# Autodesk Inventor assembly: New_Case
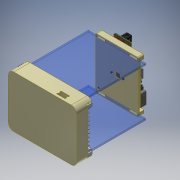
[picture p0: Inventor's stored thumbnail of the model, 180x180]
Saved by Autodesk Inventor 2017 (Build 210142000, 142)
## iProperties
Created: 2017-11-02
Part Number: New_Case
Document SubType Name: Assembly
Designer: P. Baesso
Author: P. Baesso
## Documents named in this file (16)
- E:\Rymapt_projects\Ethoscope\ethoscope_hardware\Assembled\New_Case.iam
- E:\Rymapt_projects\Ethoscope\ethoscope_hardware\core\RPi3\RPi3_ModelB.ipt
- E:\Rymapt_projects\Ethoscope\ethoscope_hardware\core_Rymapt\PiCase\lowerPiCase_small.ipt
- E:\Rymapt_projects\Ethoscope\ethoscope_hardware\core\RPi3\RasPi_Camera.ipt
- E:\Rymapt_projects\Ethoscope\ethoscope_hardware\Shield\Files\PCB_R2D2.iam
- E:\Rymapt_projects\Ethoscope\ethoscope_hardware\core_Rymapt\PiCase\upperPiCase_small.ipt
- E:\Rymapt_projects\Ethoscope\ethoscope_hardware\core_Rymapt\LightBox\sideWall_R3.ipt
- E:\Rymapt_projects\Ethoscope\ethoscope_hardware\extra\IRFilter\FB700-10-Step.ipt
- E:\Rymapt_projects\Ethoscope\ethoscope_hardware\extra\IRFilter\FilterHolder.ipt
- E:\Rymapt_projects\Ethoscope\ethoscope_hardware\core_Rymapt\LightBox\core_lightBox_R2.ipt
- E:\Rymapt_projects\Ethoscope\ethoscope_hardware\core_Rymapt\LightBox\core_lightStrip_R.ipt
- E:\Rymapt_projects\Ethoscope\ethoscope_hardware\arenas\arena_10x1_longTubes\arena_10x1_longTubes.ipt
- E:\Rymapt_projects\Ethoscope\ethoscope_hardware\extra\Screws\SpacerShiel.ipt
- E:\Rymapt_projects\Ethoscope\ethoscope_hardware\extra\Screws\M2_phillip_8mm.ipt
- E:\Rymapt_projects\Ethoscope\ethoscope_hardware\extra\IRFilter\FilterHolderSmall.ipt
- E:\Rymapt_projects\Ethoscope\ethoscope_hardware\extra\Connectors\022012021.ipt
## Components (28 placed, 16 different names)
1. arena_10x1_longTubes:1 — Mate:21, Mate:22, Mate:26
2. core_lightStrip_R:1 — Mate:24, Mate:23, Mate:25
3. core_lightBox_R2:1 — Mate:18, Mate:19, Mate:20, Mate:21, Mate:22, Mate:24, Mate:23, Mate:25, Mate:26
4. sideWall_R3:1 — Mate:7, Mate:8, Mate:9
5. sideWall_R3:2 — Mate:10, Mate:11, Mate:12, Mate:18, Mate:19, Mate:20
6. 022012021:1 — Mate:54, Flush:10, Mate:55
7. 022012021:2 — Mate:56, Flush:11, Mate:57
8. SpacerShiel:1 — Flush:9
9. M2_phillip_8mm:1 — Mate:27, Mate:28
10. M2_phillip_8mm:2 — Mate:31, Mate:34
11. M2_phillip_8mm:3 — Mate:33, Mate:36
12. M2_phillip_8mm:4 — Mate:37, Mate:38
13. M2_phillip_8mm:5 — Mate:32, Mate:35
14. M2_phillip_8mm:6 — Mate:29, Mate:30
15. RPi3_ModelB:1 — Angle:1, Angle:2, Flush:1, Flush:2, Mate:4, Flush:3, Mate:5, Flush:4, Mate:27, Mate:28, Mate:31, Mate:32, Mate:33, Mate:34, Mate:35, Mate:36
16. RasPi_Camera:1 — Mate:13, Mate:14, Mate:15, Mate:16, Mate:50, Mate:51, Mate:52, Mate:53
17. Screw_Camera — Mate:51, Mate:52
18. Screw_Camera:1 — Mate:50, Mate:53
19. PCB_R2D2:1 [sub-assembly] — Flush:3, Mate:5, Flush:4, Flush:5, Flush:9, Mate:29, Mate:30, Mate:54, Flush:10, Mate:55, Mate:56, Flush:11, Mate:57
20. lowerPiCase_small:1 — Angle:1, Angle:2, Flush:1, Flush:2, Mate:4, Flush:6, Flush:7, Mate:6, Mate:7, Mate:8, Mate:9, Mate:10, Mate:11, Mate:12, Mate:13, Mate:14, Mate:15, Mate:17, Mate:37, Mate:38, Mate:39, Mate:40, Mate:41
21. upperPiCase_small:1 — Flush:6, Flush:7, Mate:6
22. FilterHolder:1 — Flush:8
23. FB700-10-Step:1 — Mate:16, Mate:17, Flush:8
24. M2_phillip_8mm:7 — Mate:42, Mate:43
25. M2_phillip_8mm:8 — Mate:44, Mate:45
26. M2_phillip_8mm:9 — Mate:46, Mate:47
27. M2_phillip_8mm:10 — Mate:48, Mate:49
28. FilterHolderSmall:1 — Mate:39, Mate:40, Mate:41, Mate:42, Mate:43, Mate:44, Mate:45, Mate:46, Mate:47, Mate:48, Mate:49
## Relationships (67: Mate 54, Flush 11, Angle 2)
- Angle:1 (0 deg): RPi3_ModelB:1 ↔ lowerPiCase_small:1
- Angle:2 (0 deg): RPi3_ModelB:1 ↔ lowerPiCase_small:1
- Flush:1 (10.5 mm): RPi3_ModelB:1 ↔ lowerPiCase_small:1
- Flush:2: RPi3_ModelB:1 ↔ lowerPiCase_small:1
- Mate:4: RPi3_ModelB:1 ↔ lowerPiCase_small:1
- Flush:3: RPi3_ModelB:1 ↔ PCB_R2D2:1
- Mate:5 (1 mm): RPi3_ModelB:1 ↔ PCB_R2D2:1
- Flush:4: RPi3_ModelB:1 ↔ PCB_R2D2:1
- Flush:5 (1 mm): PCB_R2D2:1
- Flush:6: lowerPiCase_small:1 ↔ upperPiCase_small:1
- Flush:7: lowerPiCase_small:1 ↔ upperPiCase_small:1
- Mate:6: lowerPiCase_small:1 ↔ upperPiCase_small:1
- Mate:7: sideWall_R3:1 ↔ lowerPiCase_small:1
- Mate:8: sideWall_R3:1 ↔ lowerPiCase_small:1
- Mate:9: sideWall_R3:1 ↔ lowerPiCase_small:1
- Mate:10: sideWall_R3:2 ↔ lowerPiCase_small:1
- Mate:11: sideWall_R3:2 ↔ lowerPiCase_small:1
- Mate:12: sideWall_R3:2 ↔ lowerPiCase_small:1
- Mate:13: RasPi_Camera:1 ↔ lowerPiCase_small:1
- Mate:14: RasPi_Camera:1 ↔ lowerPiCase_small:1
- Mate:15: RasPi_Camera:1 ↔ lowerPiCase_small:1
- Mate:16: RasPi_Camera:1 ↔ FB700-10-Step:1
- Mate:17 (1 mm): lowerPiCase_small:1 ↔ FB700-10-Step:1
- Flush:8: FilterHolder:1 ↔ FB700-10-Step:1
- Mate:18: core_lightBox_R2:1 ↔ sideWall_R3:2
- Mate:19: core_lightBox_R2:1 ↔ sideWall_R3:2
- Mate:20: core_lightBox_R2:1 ↔ sideWall_R3:2
- Mate:21: arena_10x1_longTubes:1 ↔ core_lightBox_R2:1
- Mate:22: arena_10x1_longTubes:1 ↔ core_lightBox_R2:1
- Mate:24: core_lightStrip_R:1 ↔ core_lightBox_R2:1
- Mate:23: core_lightStrip_R:1 ↔ core_lightBox_R2:1
- Mate:25 (0.1 mm): core_lightStrip_R:1 ↔ core_lightBox_R2:1
- Mate:26: arena_10x1_longTubes:1 ↔ core_lightBox_R2:1
- Flush:9: SpacerShiel:1 ↔ PCB_R2D2:1
- Mate:27: M2_phillip_8mm:1 ↔ RPi3_ModelB:1
- Mate:28 (0.1 mm): M2_phillip_8mm:1 ↔ RPi3_ModelB:1
- Mate:29: M2_phillip_8mm:6 ↔ PCB_R2D2:1
- Mate:30 (0.1 mm): M2_phillip_8mm:6 ↔ PCB_R2D2:1
- Mate:31: M2_phillip_8mm:2 ↔ RPi3_ModelB:1
- Mate:32: M2_phillip_8mm:5 ↔ RPi3_ModelB:1
- Mate:33: M2_phillip_8mm:3 ↔ RPi3_ModelB:1
- Mate:34 (0.1 mm): M2_phillip_8mm:2 ↔ RPi3_ModelB:1
- Mate:35 (0.1 mm): M2_phillip_8mm:5 ↔ RPi3_ModelB:1
- Mate:36 (0.1 mm): M2_phillip_8mm:3 ↔ RPi3_ModelB:1
- Mate:37: M2_phillip_8mm:4 ↔ lowerPiCase_small:1
- Mate:38 (0.1 mm): M2_phillip_8mm:4 ↔ lowerPiCase_small:1
- Mate:39: lowerPiCase_small:1 ↔ FilterHolderSmall:1
- Mate:40: lowerPiCase_small:1 ↔ FilterHolderSmall:1
- Mate:41: lowerPiCase_small:1 ↔ FilterHolderSmall:1
- Mate:42: M2_phillip_8mm:7 ↔ FilterHolderSmall:1
- Mate:43 (0.1 mm): M2_phillip_8mm:7 ↔ FilterHolderSmall:1
- Mate:44: M2_phillip_8mm:8 ↔ FilterHolderSmall:1
- Mate:45 (0.1 mm): M2_phillip_8mm:8 ↔ FilterHolderSmall:1
- Mate:46: M2_phillip_8mm:9 ↔ FilterHolderSmall:1
- Mate:47 (0.1 mm): M2_phillip_8mm:9 ↔ FilterHolderSmall:1
- Mate:48: M2_phillip_8mm:10 ↔ FilterHolderSmall:1
- Mate:49 (0.1 mm): M2_phillip_8mm:10 ↔ FilterHolderSmall:1
- Mate:50: RasPi_Camera:1 ↔ Screw_Camera:1
- Mate:51: RasPi_Camera:1 ↔ Screw_Camera
- Mate:52 (0.1 mm): RasPi_Camera:1 ↔ Screw_Camera
- Mate:53 (0.1 mm): RasPi_Camera:1 ↔ Screw_Camera:1
- Mate:54: 022012021:1 ↔ PCB_R2D2:1
- Flush:10 (-0.254 mm): 022012021:1 ↔ PCB_R2D2:1
- Mate:55 (0.1 mm): 022012021:1 ↔ PCB_R2D2:1
- Mate:56: 022012021:2 ↔ PCB_R2D2:1
- Flush:11 (-0.254 mm): 022012021:2 ↔ PCB_R2D2:1
- Mate:57 (0.1 mm): 022012021:2 ↔ PCB_R2D2:1
